# Autodesk Inventor assembly: frame_1_0
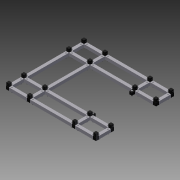
[picture p0: Inventor's stored thumbnail of the model, 180x180]
Saved by Autodesk Inventor 2011 (Build 150239000, 239)
## iProperties
Created: 2013-01-19
Part Number: frame_1_0
Document SubType Name: Assembly
Designer: Christopher
Author: Christopher
## Documents named in this file (27)
- F:\Users\Christopher\Documents\GitHub\2013CAD\2013 robot\forklift\robot_frame\tubes_layer2\frame_level1_temp.iam
- F:\Users\Christopher\Documents\GitHub\2013CAD\2013 robot\forklift\Misc parts\3-way corner.ipt
- F:\Users\Christopher\Documents\GitHub\2013CAD\2013 robot\forklift\Misc parts\4-way corner.ipt
- F:\Users\Christopher\Documents\GitHub\2013CAD\2013 robot\forklift\Misc parts\5-way corner.ipt
- F:\Users\Christopher\Documents\GitHub\2013CAD\2013 robot\forklift\Misc parts\1.5_bolt_.25_20.ipt
- F:\Users\Christopher\Documents\GitHub\2013CAD\2013 robot\forklift\robot_frame\tubes_layer2\tube_m_b_in_cross.ipt
- F:\Users\Christopher\Documents\GitHub\2013CAD\2013 robot\forklift\robot_frame\tubes_layer2\tube_m_r_in_mid.ipt
- F:\Users\Christopher\Documents\GitHub\2013CAD\2013 robot\forklift\robot_frame\tubes_layer2\tube_r_b_in.ipt
- F:\Users\Christopher\Documents\GitHub\2013CAD\2013 robot\forklift\robot_frame\tubes_layer2\tube_r_f_in.ipt
- F:\Users\Christopher\Documents\GitHub\2013CAD\2013 robot\forklift\robot_frame\tubes_layer2\tube_m_r_out_center.ipt
- F:\Users\Christopher\Documents\GitHub\2013CAD\2013 robot\forklift\robot_frame\tubes_layer2\tube_b_r_in_wheel.ipt
- F:\Users\Christopher\Documents\GitHub\2013CAD\2013 robot\forklift\robot_frame\tubes_layer2\tube_r_b_out.ipt
- F:\Users\Christopher\Documents\GitHub\2013CAD\2013 robot\forklift\robot_frame\tubes_layer2\tube_b_r_wheel.ipt
- F:\Users\Christopher\Documents\GitHub\2013CAD\2013 robot\forklift\robot_frame\tubes_layer2\tube_f_r_in_wheel.ipt
- F:\Users\Christopher\Documents\GitHub\2013CAD\2013 robot\forklift\robot_frame\tubes_layer2\tube_f_r_out_wheel.ipt
- F:\Users\Christopher\Documents\GitHub\2013CAD\2013 robot\forklift\robot_frame\tubes_layer2\tube_r_f_out.ipt
- F:\Users\Christopher\Documents\GitHub\2013CAD\2013 robot\forklift\robot_frame\tubes_layer2\tube_m_b_out_back.ipt
- F:\Users\Christopher\Documents\GitHub\2013CAD\2013 robot\forklift\robot_frame\tubes_layer1\tube_b_l_in_wheel.ipt
- F:\Users\Christopher\Documents\GitHub\2013CAD\2013 robot\forklift\robot_frame\tubes_layer1\tube_m_l_in.ipt
- F:\Users\Christopher\Documents\GitHub\2013CAD\2013 robot\forklift\robot_frame\tubes_layer1\tube_f_l_in_wheel.ipt
- F:\Users\Christopher\Documents\GitHub\2013CAD\2013 robot\forklift\robot_frame\tubes_layer1\tube_l_f_out.ipt
- F:\Users\Christopher\Documents\GitHub\2013CAD\2013 robot\forklift\robot_frame\tubes_layer1\tube_l_f_in.ipt
- F:\Users\Christopher\Documents\GitHub\2013CAD\2013 robot\forklift\robot_frame\tubes_layer1\tube_l_b_in.ipt
- F:\Users\Christopher\Documents\GitHub\2013CAD\2013 robot\forklift\robot_frame\tubes_layer1\tube_l_b_out.ipt
- F:\Users\Christopher\Documents\GitHub\2013CAD\2013 robot\forklift\robot_frame\tubes_layer1\tube_b_l_out_wheel.ipt
- F:\Users\Christopher\Documents\GitHub\2013CAD\2013 robot\forklift\robot_frame\tubes_layer1\tube_f_l_out_wheel.ipt
- F:\Users\Christopher\Documents\GitHub\2013CAD\2013 robot\forklift\robot_frame\tubes_layer1\tube_m_l_out.ipt
## Components (84 placed, 26 different names)
1. 5-way corner:2 — Mate:4, Insert:5, Mate:8, Insert:13, Mate:18, Insert:35
2. 1.5_bolt_.25_20:1
3. 5-way corner:3 — Mate:5, Insert:7, Mate:6, Insert:9, Mate:7, Insert:11, Mate:12, Insert:23
4. 1.5_bolt_.25_20:2
5. 5-way corner:4 — Mate:30, Insert:58, Mate:31, Insert:62, Mate:34, Insert:70
6. 1.5_bolt_.25_20:3 — Insert:12
7. tube_m_b_in_cross:1 — Mate:6, Insert:9, Insert:10, Mate:25, Insert:49, Insert:51
8. tube_m_r_in_mid:1 — Mate:4, Insert:5, Insert:6, Mate:5, Insert:7, Insert:8
9. 1.5_bolt_.25_20:4 — Insert:6
10. 1.5_bolt_.25_20:5 — Insert:22
11. 1.5_bolt_.25_20:6 — Insert:26
12. 1.5_bolt_.25_20:7 — Insert:28
13. 1.5_bolt_.25_20:8 — Insert:30
14. 1.5_bolt_.25_20:10 — Insert:8
15. 1.5_bolt_.25_20:11 — Insert:10
16. 1.5_bolt_.25_20:12 — Insert:14
17. 1.5_bolt_.25_20:13 — Insert:16
18. 1.5_bolt_.25_20:14 — Insert:18
19. 1.5_bolt_.25_20:15 — Insert:19
20. 1.5_bolt_.25_20:16 — Insert:24
21. tube_r_b_in:1 — Mate:7, Insert:11, Insert:12, Mate:11, Insert:19, Insert:20
22. tube_r_f_in:1 — Mate:8, Insert:13, Insert:14, Mate:9, Insert:15, Insert:16
23. tube_m_r_out_center:1 — Mate:10, Insert:17, Insert:18, Insert:21, Flush:1, Insert:22
24. 4-way corner:2 — Mate:9, Insert:15, Mate:10, Insert:17, Mate:20, Insert:39
25. 4-way corner:3 — Mate:11, Insert:20, Insert:21, Flush:1, Mate:17, Insert:32
26. 3-way corner:2 — Mate:15, Insert:29, Mate:16, Insert:31
27. 4-way corner:4 — Mate:13, Insert:25, Mate:14, Insert:27, Mate:24, Insert:47
28. tube_b_r_in_wheel:1 — Mate:12, Insert:23, Insert:24, Mate:13, Insert:25, Insert:26
29. tube_r_b_out:1 — Mate:14, Insert:27, Insert:28, Mate:15, Insert:29, Insert:30
30. 1.5_bolt_.25_20:17 — Insert:48
31. 1.5_bolt_.25_20:18 — Insert:56
32. 1.5_bolt_.25_20:19 — Insert:42
33. 1.5_bolt_.25_20:20 — Insert:40
34. 1.5_bolt_.25_20:21 — Insert:36
35. 1.5_bolt_.25_20:22 — Insert:51
36. 1.5_bolt_.25_20:23 — Insert:52
37. 1.5_bolt_.25_20:24 — Insert:33
38. 1.5_bolt_.25_20:25 — Insert:45
39. 1.5_bolt_.25_20:26 — Insert:38
40. 1.5_bolt_.25_20:27 — Insert:46
41. 1.5_bolt_.25_20:28 — Insert:34
42. tube_b_r_wheel:1 — Mate:16, Mate:17, Insert:31, Insert:32, Insert:33, Insert:34
43. tube_f_r_in_wheel:1 — Mate:18, Insert:35, Insert:36, Mate:19, Insert:37, Insert:38
44. tube_f_r_out_wheel:1 — Mate:20, Insert:39, Insert:40, Mate:21, Insert:41, Insert:42
45. 3-way corner:3 — Mate:21, Insert:41, Mate:23, Insert:43
46. 3-way corner:4 — Mate:19, Insert:37, Mate:22, Insert:44
47. tube_r_f_out:1 — Mate:22, Mate:23, Insert:43, Insert:44, Insert:45, Insert:46
48. tube_m_b_out_back:1 — Mate:24, Insert:47, Insert:48, Insert:52, Mate:26, Insert:53
49. 5-way corner:5 — Mate:25, Insert:49, Mate:27, Insert:55, Mate:29, Insert:59, Mate:35, Insert:71
50. 4-way corner:5 — Mate:26, Insert:53, Mate:28, Insert:54, Mate:36, Insert:72
51. tube_b_l_in_wheel:1 — Mate:27, Mate:28, Insert:54, Insert:55, Insert:56, Insert:57
52. 1.5_bolt_.25_20:30 — Insert:67
53. 1.5_bolt_.25_20:31 — Insert:69
54. 1.5_bolt_.25_20:32 — Insert:79
55. 1.5_bolt_.25_20:33 — Insert:78
56. 1.5_bolt_.25_20:34 — Insert:63
57. 1.5_bolt_.25_20:35 — Insert:57
58. 1.5_bolt_.25_20:36 — Insert:66
59. 1.5_bolt_.25_20:37 — Insert:61
60. 1.5_bolt_.25_20:38 — Insert:60
61. tube_m_l_in:1 — Mate:29, Mate:30, Insert:58, Insert:59, Insert:60, Insert:61
62. tube_f_l_in_wheel:1 — Mate:31, Insert:62, Insert:63, Mate:32, Insert:64, Insert:67
63. 3-way corner:5 — Mate:32, Insert:64, Flush:2, Insert:65
64. tube_l_f_out:1 — Flush:2, Insert:65, Insert:66, Mate:33, Insert:68, Insert:69
65. 3-way corner:6 — Mate:33, Insert:68, Mate:42, Insert:83
66. tube_l_f_in:1 — Mate:34, Insert:70, Flush:3, Insert:73, Insert:76, Insert:77
67. tube_l_b_in:1 — Mate:35, Insert:71, Flush:4, Insert:74, Insert:78, Insert:93
68. tube_l_b_out:1 — Mate:36, Insert:72, Flush:5, Insert:75, Insert:79, Insert:80
69. 4-way corner:6 — Flush:3, Insert:73, Mate:40, Mate:41, Insert:84, Insert:85
70. 4-way corner:7 — Flush:4, Insert:74, Mate:38, Insert:81, Mate:39, Insert:86, Insert:87
71. 3-way corner:7 — Flush:5, Insert:75, Mate:37, Insert:82, Insert:88
72. 1.5_bolt_.25_20:39 — Insert:76
73. 1.5_bolt_.25_20:40 — Insert:80
74. 1.5_bolt_.25_20:41 — Insert:77
75. 1.5_bolt_.25_20:42 — Insert:93
76. 1.5_bolt_.25_20:43 — Insert:91
77. 1.5_bolt_.25_20:44 — Insert:92
78. 1.5_bolt_.25_20:45 — Insert:90
79. 1.5_bolt_.25_20:46 — Insert:89
80. tube_b_l_out_wheel:1 — Mate:37, Mate:38, Insert:81, Insert:82, Insert:87, Insert:88, Insert:94, Insert:95
81. tube_f_l_out_wheel:1 — Mate:41, Mate:42, Insert:83, Insert:84, Insert:89, Insert:90
82. tube_m_l_out:1 — Mate:39, Mate:40, Insert:85, Insert:86, Insert:91, Insert:92
83. 1.5_bolt_.25_20:50 — Insert:94
84. 1.5_bolt_.25_20:51 — Insert:95
## Relationships (134: Insert 90, Mate 39, Flush 5)
- Mate:4: 5-way corner:2 ↔ tube_m_r_in_mid:1
- Insert:5: 5-way corner:2 ↔ tube_m_r_in_mid:1
- Insert:6: tube_m_r_in_mid:1 ↔ 1.5_bolt_.25_20:4
- Mate:5: 5-way corner:3 ↔ tube_m_r_in_mid:1
- Insert:7: 5-way corner:3 ↔ tube_m_r_in_mid:1
- Insert:8: tube_m_r_in_mid:1 ↔ 1.5_bolt_.25_20:10
- Mate:6: 5-way corner:3 ↔ tube_m_b_in_cross:1
- Insert:9: 5-way corner:3 ↔ tube_m_b_in_cross:1
- Insert:10: tube_m_b_in_cross:1 ↔ 1.5_bolt_.25_20:11
- Mate:7: 5-way corner:3 ↔ tube_r_b_in:1
- Insert:11: 5-way corner:3 ↔ tube_r_b_in:1
- Insert:12: 1.5_bolt_.25_20:3 ↔ tube_r_b_in:1
- Mate:8: 5-way corner:2 ↔ tube_r_f_in:1
- Insert:13: 5-way corner:2 ↔ tube_r_f_in:1
- Insert:14: 1.5_bolt_.25_20:12 ↔ tube_r_f_in:1
- Mate:9: tube_r_f_in:1 ↔ 4-way corner:2
- Insert:15: tube_r_f_in:1 ↔ 4-way corner:2
- Mate:10: tube_m_r_out_center:1 ↔ 4-way corner:2
- Insert:16: 1.5_bolt_.25_20:13 ↔ tube_r_f_in:1
- Insert:17: tube_m_r_out_center:1 ↔ 4-way corner:2
- Insert:18: 1.5_bolt_.25_20:14 ↔ tube_m_r_out_center:1
- Mate:11: tube_r_b_in:1 ↔ 4-way corner:3
- Insert:19: 1.5_bolt_.25_20:15 ↔ tube_r_b_in:1
- Insert:20: tube_r_b_in:1 ↔ 4-way corner:3
- Insert:21: tube_m_r_out_center:1 ↔ 4-way corner:3
- Flush:1: tube_m_r_out_center:1 ↔ 4-way corner:3
- Insert:22: 1.5_bolt_.25_20:5 ↔ tube_m_r_out_center:1
- Mate:12: 5-way corner:3 ↔ tube_b_r_in_wheel:1
- Insert:23: 5-way corner:3 ↔ tube_b_r_in_wheel:1
- Insert:24: 1.5_bolt_.25_20:16 ↔ tube_b_r_in_wheel:1
- Mate:13: 4-way corner:4 ↔ tube_b_r_in_wheel:1
- Insert:25: 4-way corner:4 ↔ tube_b_r_in_wheel:1
- Insert:26: 1.5_bolt_.25_20:6 ↔ tube_b_r_in_wheel:1
- Mate:14: 4-way corner:4 ↔ tube_r_b_out:1
- Insert:27: 4-way corner:4 ↔ tube_r_b_out:1
- Insert:28: 1.5_bolt_.25_20:7 ↔ tube_r_b_out:1
- Mate:15: 3-way corner:2 ↔ tube_r_b_out:1
- Insert:29: 3-way corner:2 ↔ tube_r_b_out:1
- Insert:30: 1.5_bolt_.25_20:8 ↔ tube_r_b_out:1
- Mate:16: 3-way corner:2 ↔ tube_b_r_wheel:1
- Mate:17: 4-way corner:3 ↔ tube_b_r_wheel:1
- Insert:31: 3-way corner:2 ↔ tube_b_r_wheel:1
- Insert:32: 4-way corner:3 ↔ tube_b_r_wheel:1
- Insert:33: 1.5_bolt_.25_20:24 ↔ tube_b_r_wheel:1
- Insert:34: 1.5_bolt_.25_20:28 ↔ tube_b_r_wheel:1
- Mate:18: 5-way corner:2 ↔ tube_f_r_in_wheel:1
- Insert:35: 5-way corner:2 ↔ tube_f_r_in_wheel:1
- Insert:36: 1.5_bolt_.25_20:21 ↔ tube_f_r_in_wheel:1
- Mate:19: tube_f_r_in_wheel:1 ↔ 3-way corner:4
- Insert:37: tube_f_r_in_wheel:1 ↔ 3-way corner:4
- Insert:38: 1.5_bolt_.25_20:26 ↔ tube_f_r_in_wheel:1
- Mate:20: 4-way corner:2 ↔ tube_f_r_out_wheel:1
- Insert:39: 4-way corner:2 ↔ tube_f_r_out_wheel:1
- Insert:40: 1.5_bolt_.25_20:20 ↔ tube_f_r_out_wheel:1
- Mate:21: tube_f_r_out_wheel:1 ↔ 3-way corner:3
- Insert:41: tube_f_r_out_wheel:1 ↔ 3-way corner:3
- Insert:42: 1.5_bolt_.25_20:19 ↔ tube_f_r_out_wheel:1
- Mate:22: 3-way corner:4 ↔ tube_r_f_out:1
- Mate:23: 3-way corner:3 ↔ tube_r_f_out:1
- Insert:43: 3-way corner:3 ↔ tube_r_f_out:1
- Insert:44: 3-way corner:4 ↔ tube_r_f_out:1
- Insert:45: 1.5_bolt_.25_20:25 ↔ tube_r_f_out:1
- Insert:46: 1.5_bolt_.25_20:27 ↔ tube_r_f_out:1
- Mate:24: 4-way corner:4 ↔ tube_m_b_out_back:1
- Insert:47: 4-way corner:4 ↔ tube_m_b_out_back:1
- Insert:48: 1.5_bolt_.25_20:17 ↔ tube_m_b_out_back:1
- Mate:25: tube_m_b_in_cross:1 ↔ 5-way corner:5
- Insert:49: tube_m_b_in_cross:1 ↔ 5-way corner:5
- Insert:51: tube_m_b_in_cross:1 ↔ 1.5_bolt_.25_20:22
- Insert:52: 1.5_bolt_.25_20:23 ↔ tube_m_b_out_back:1
- Mate:26: tube_m_b_out_back:1 ↔ 4-way corner:5
- Insert:53: tube_m_b_out_back:1 ↔ 4-way corner:5
- Mate:27: 5-way corner:5 ↔ tube_b_l_in_wheel:1
- Mate:28: 4-way corner:5 ↔ tube_b_l_in_wheel:1
- Insert:54: 4-way corner:5 ↔ tube_b_l_in_wheel:1
- Insert:55: 5-way corner:5 ↔ tube_b_l_in_wheel:1
- Insert:56: 1.5_bolt_.25_20:18 ↔ tube_b_l_in_wheel:1
- Insert:57: tube_b_l_in_wheel:1 ↔ 1.5_bolt_.25_20:35
- Mate:29: 5-way corner:5 ↔ tube_m_l_in:1
- Mate:30: 5-way corner:4 ↔ tube_m_l_in:1
- Insert:58: 5-way corner:4 ↔ tube_m_l_in:1
- Insert:59: 5-way corner:5 ↔ tube_m_l_in:1
- Insert:60: 1.5_bolt_.25_20:38 ↔ tube_m_l_in:1
- Insert:61: 1.5_bolt_.25_20:37 ↔ tube_m_l_in:1
- Mate:31: 5-way corner:4 ↔ tube_f_l_in_wheel:1
- Insert:62: 5-way corner:4 ↔ tube_f_l_in_wheel:1
- Insert:63: 1.5_bolt_.25_20:34 ↔ tube_f_l_in_wheel:1
- Mate:32: tube_f_l_in_wheel:1 ↔ 3-way corner:5
- Insert:64: tube_f_l_in_wheel:1 ↔ 3-way corner:5
- Flush:2: 3-way corner:5 ↔ tube_l_f_out:1
- Insert:65: 3-way corner:5 ↔ tube_l_f_out:1
- Insert:66: 1.5_bolt_.25_20:36 ↔ tube_l_f_out:1
- Insert:67: 1.5_bolt_.25_20:30 ↔ tube_f_l_in_wheel:1
- Mate:33: tube_l_f_out:1 ↔ 3-way corner:6
- Insert:68: tube_l_f_out:1 ↔ 3-way corner:6
- Insert:69: 1.5_bolt_.25_20:31 ↔ tube_l_f_out:1
- Mate:34: 5-way corner:4 ↔ tube_l_f_in:1
- Mate:35: 5-way corner:5 ↔ tube_l_b_in:1
- Mate:36: 4-way corner:5 ↔ tube_l_b_out:1
- Insert:70: 5-way corner:4 ↔ tube_l_f_in:1
- Insert:71: 5-way corner:5 ↔ tube_l_b_in:1
- Insert:72: 4-way corner:5 ↔ tube_l_b_out:1
- Flush:3: tube_l_f_in:1 ↔ 4-way corner:6
- Flush:4: tube_l_b_in:1 ↔ 4-way corner:7
- Flush:5: tube_l_b_out:1 ↔ 3-way corner:7
- Insert:73: tube_l_f_in:1 ↔ 4-way corner:6
- Insert:74: tube_l_b_in:1 ↔ 4-way corner:7
- Insert:75: tube_l_b_out:1 ↔ 3-way corner:7
- Insert:76: tube_l_f_in:1 ↔ 1.5_bolt_.25_20:39
- Insert:77: tube_l_f_in:1 ↔ 1.5_bolt_.25_20:41
- Insert:78: 1.5_bolt_.25_20:33 ↔ tube_l_b_in:1
- Insert:79: 1.5_bolt_.25_20:32 ↔ tube_l_b_out:1
- Insert:80: tube_l_b_out:1 ↔ 1.5_bolt_.25_20:40
- Mate:37: 3-way corner:7 ↔ tube_b_l_out_wheel:1
- Mate:38: 4-way corner:7 ↔ tube_b_l_out_wheel:1
- Insert:81: 4-way corner:7 ↔ tube_b_l_out_wheel:1
- Insert:82: 3-way corner:7 ↔ tube_b_l_out_wheel:1
- Mate:39: 4-way corner:7 ↔ tube_m_l_out:1
- Mate:40: 4-way corner:6 ↔ tube_m_l_out:1
- Mate:41: 4-way corner:6 ↔ tube_f_l_out_wheel:1
- Mate:42: 3-way corner:6 ↔ tube_f_l_out_wheel:1
- Insert:83: 3-way corner:6 ↔ tube_f_l_out_wheel:1
- Insert:84: 4-way corner:6 ↔ tube_f_l_out_wheel:1
- Insert:85: 4-way corner:6 ↔ tube_m_l_out:1
- Insert:86: 4-way corner:7 ↔ tube_m_l_out:1
- Insert:87: 4-way corner:7 ↔ tube_b_l_out_wheel:1
- Insert:88: 3-way corner:7 ↔ tube_b_l_out_wheel:1
- Insert:89: 1.5_bolt_.25_20:46 ↔ tube_f_l_out_wheel:1
- Insert:90: 1.5_bolt_.25_20:45 ↔ tube_f_l_out_wheel:1
- Insert:91: 1.5_bolt_.25_20:43 ↔ tube_m_l_out:1
- Insert:92: 1.5_bolt_.25_20:44 ↔ tube_m_l_out:1
- Insert:93: tube_l_b_in:1 ↔ 1.5_bolt_.25_20:42
- Insert:94: tube_b_l_out_wheel:1 ↔ 1.5_bolt_.25_20:50
- Insert:95: tube_b_l_out_wheel:1 ↔ 1.5_bolt_.25_20:51
